# Autodesk Inventor assembly: Model
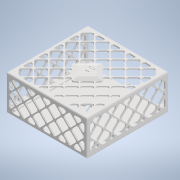
[picture p0: Inventor's stored thumbnail of the model, 180x180]
Saved by Autodesk Inventor 2020 (Build 240168000, 168)
## iProperties
Created: 2020-06-10
Part Number: Model
Document SubType Name: Assembly
Designer: maple
Author: maple
## Documents named in this file (6)
- C:\Users\maple\Desktop\Model.iam
- C:\Users\maple\Desktop\Face.ipt
- C:\Users\maple\Desktop\Side L.ipt
- C:\Users\maple\Desktop\Side R.ipt
- C:\Users\maple\Desktop\Back.ipt
- C:\Users\maple\Desktop\All.ipt
## Components (5 placed, 5 different names)
1. All:1 — Mate:1, Flush:1, Mate:2, Mate:3, Mate:5, Mate:6, Mate:8, Mate:9, Mate:11
2. Face:1 — Mate:1, Flush:1, Mate:2, Mate:4, Mate:7
3. Side L:1 — Mate:3, Mate:4, Mate:5
4. Side R:1 — Mate:6, Mate:7, Mate:8, Mate:10
5. Back:1 — Mate:9, Mate:10, Mate:11
## Relationships (12: Mate 11, Flush 1)
- Mate:1: All:1 ↔ Face:1
- Flush:1: All:1 ↔ Face:1
- Mate:2: All:1 ↔ Face:1
- Mate:3: All:1 ↔ Side L:1
- Mate:4: Face:1 ↔ Side L:1
- Mate:5: All:1 ↔ Side L:1
- Mate:6: All:1 ↔ Side R:1
- Mate:7: Face:1 ↔ Side R:1
- Mate:8: All:1 ↔ Side R:1
- Mate:9: All:1 ↔ Back:1
- Mate:10: Side R:1 ↔ Back:1
- Mate:11: All:1 ↔ Back:1
